# Autodesk Inventor assembly: main climber
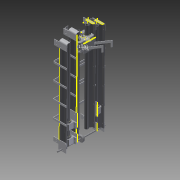
[picture p0: Inventor's stored thumbnail of the model, 180x180]
Saved by Autodesk Inventor 2013 (Build 170138000, 138)
## iProperties
Created: 2013-01-25
Part Number: main climber
Document SubType Name: Assembly
Designer: Arpan
Mass: 3389.77 g
Surface Area: 12723.3 cm^2
Volume: 2953.27 cm^3
Density: 1.1478 g/cm^3
Author: Arpan
## Documents named in this file (18)
- C:\Users\Arpan\Documents\GitHub\frc2013CAD\Cimber actual\main climber.iam
- C:\Users\Arpan\Documents\GitHub\frc2013CAD\Cimber actual\Shaft 26 inch.ipt
- C:\Users\Arpan\Documents\GitHub\frc2013CAD\Cimber actual\Bearing Block long style.iam
- C:\Users\Arpan\Documents\GitHub\frc2013CAD\Cimber actual\hook mount plate.ipt
- C:\Users\Arpan\Documents\GitHub\frc2013CAD\Cimber actual\tie-together tier 1.ipt
- C:\Users\Arpan\Documents\GitHub\frc2013CAD\Cimber actual\endstop.ipt
- C:\Users\Arpan\Documents\GitHub\frc2013CAD\Cimber actual\hook faceplate.ipt
- C:\Users\Arpan\Documents\GitHub\frc2013CAD\Cimber actual\hook.ipt
- C:\Users\Arpan\Documents\GitHub\frc2013CAD\Cimber actual\face mount.ipt
- C:\Users\Arpan\Documents\GitHub\frc2013CAD\Cimber actual\bearing block short style.iam
- C:\Users\Arpan\Documents\GitHub\frc2013CAD\Cimber actual\upper face mount.ipt
- C:\Users\Arpan\Documents\GitHub\frc2013CAD\Cimber actual\tie-together tier 2.ipt
- C:\Users\Arpan\Documents\GitHub\frc2013CAD\Cimber actual\arm mout.ipt
- C:\Users\Arpan\Documents\GitHub\frc2013CAD\Cimber actual\14 inch shaft.ipt
- C:\Users\Arpan\Documents\GitHub\frc2013CAD\Cimber actual\rough pulley.ipt
- C:\Users\Arpan\Documents\GitHub\frc2013CAD\Cimber actual\hook mount plate 2.ipt
- C:\Users\Arpan\Documents\GitHub\frc2013CAD\Cimber actual\endstop 2.ipt
- C:\Users\Arpan\Documents\GitHub\frc2013CAD\Cimber actual\pulley mount.ipt
## Components (36 placed, 17 different names)
1. Shaft 26 inch:1 — Flush:1, Angle:1, Mate:2, Flush:2, Angle:2, Mate:25, Mate:26, Mate:27, Mate:28, Mate:29, Mate:30, Mate:31, Mate:32, Mate:33, Mate:38, Mate:39, Mate:40, Mate:103, Flush:31, Mate:104, Mate:109, Mate:110, Mate:111
2. Shaft 26 inch:2 — Flush:1, Angle:1, Mate:1, Flush:2, Flush:7, Mate:10, Mate:11, Mate:37, Flush:15, Flush:16, Mate:48, Mate:106, Mate:107
3. Bearing Block long style:1 [sub-assembly] — Mate:1, Mate:3, Flush:3
4. Bearing Block long style:2 [sub-assembly] — Mate:2, Mate:3, Angle:2, Flush:3, Mate:98, Flush:25, Flush:26
5. hook mount plate:1 — Mate:98, Mate:99, Flush:25, Flush:26, Flush:27, Mate:100, Flush:28, Mate:101, Flush:29
6. endstop:2 — Flush:7, Mate:10, Mate:11, Mate:116, Flush:35, Flush:36
7. hook faceplate:1 — Mate:20, Mate:21, Mate:22, Flush:13, Flush:14, Mate:23, Mate:99, Mate:101, Flush:29, Mate:102, Flush:30
8. hook:1 — Mate:22, Flush:14, Mate:102
9. hook:2 — Mate:20, Mate:21, Flush:13, Mate:23
10. tie-together tier 1:1 — Mate:25, Mate:26, Mate:27
11. tie-together tier 1:2 — Mate:28, Mate:29, Mate:30
12. tie-together tier 1:3 — Mate:31, Mate:32, Mate:33
13. face mount:1 — Mate:37, Flush:15, Flush:16, Mate:43, Mate:84, Mate:85, Mate:118, Flush:37, Flush:38
14. face mount:2 — Mate:38, Mate:39, Mate:40
15. bearing block short style:2 [sub-assembly] — Mate:43, Flush:19, Mate:84, Mate:85, Flush:23
16. bearing block short style:3 [sub-assembly] — Mate:64, Angle:3, Mate:105
17. bearing block short style:4 [sub-assembly] — Mate:48, Flush:19, Mate:65, Mate:108
18. Shaft 26 inch:3 — Mate:65, Angle:4, Flush:20, Mate:67, Mate:68, Flush:22, Mate:78, Mate:79, Mate:80, Mate:82, Mate:83, Flush:23, Mate:88, Mate:89, Mate:117
19. Shaft 26 inch:4 — Mate:64, Angle:3, Angle:4, Flush:20, Mate:76, Mate:77, Mate:86, Mate:87, Mate:90, Mate:91, Mate:112, Mate:113, Mate:114
20. endstop:3 — Mate:67, Mate:68, Flush:22
21. tie-together tier 2:2 — Mate:76, Mate:77, Mate:78, Mate:117
22. tie-together tier 2:3 — Mate:79, Mate:80
23. tie-together tier 2:4 — Mate:82, Mate:83
24. tie-together tier 2:5 — Mate:86, Mate:87
25. arm mout:1 — Mate:90, Mate:91, Mate:92
26. arm mout:2 — Mate:88, Mate:89, Flush:24, Mate:96
27. 14 inch shaft:1 — Mate:92, Flush:24, Mate:93
28. rough pulley:1 — Mate:93, Mate:96
29. hook mount plate 2:1 — Flush:27, Mate:100, Flush:28, Flush:30
30. upper face mount:1 — Mate:103, Flush:31, Mate:104, Mate:105
31. upper face mount:2 — Mate:106, Mate:107, Mate:108
32. endstop 2:1 — Mate:112, Mate:113, Mate:114, Mate:115, Flush:33, Flush:34
33. endstop 2:2 — Mate:109, Mate:110, Mate:111
34. pulley mount:2 — Mate:115, Flush:33, Flush:34
35. pulley mount:3 — Mate:116, Flush:35, Flush:36
36. pulley mount:4 — Mate:118, Flush:37, Flush:38
## Relationships (97: Mate 67, Flush 26, Angle 4)
- Flush:1: Shaft 26 inch:1 ↔ Shaft 26 inch:2
- Angle:1 (180 deg): Shaft 26 inch:1 ↔ Shaft 26 inch:2
- Mate:1: Shaft 26 inch:2 ↔ Bearing Block long style:1
- Mate:2: Shaft 26 inch:1 ↔ Bearing Block long style:2
- Mate:3 (12.7 mm): Bearing Block long style:1 ↔ Bearing Block long style:2
- Flush:2: Shaft 26 inch:1 ↔ Shaft 26 inch:2
- Angle:2 (0 deg): Shaft 26 inch:1 ↔ Bearing Block long style:2
- Flush:3: Bearing Block long style:1 ↔ Bearing Block long style:2
- Flush:7: Shaft 26 inch:2 ↔ endstop:2
- Mate:10: Shaft 26 inch:2 ↔ endstop:2
- Mate:11: Shaft 26 inch:2 ↔ endstop:2
- Mate:20: hook faceplate:1 ↔ hook:2
- Mate:21 (-26.1747 mm): hook faceplate:1 ↔ hook:2
- Mate:22 (26.1874 mm): hook faceplate:1 ↔ hook:1
- Flush:13 (6.35 mm): hook faceplate:1 ↔ hook:2
- Flush:14 (6.35 mm): hook faceplate:1 ↔ hook:1
- Mate:23 (26.1658 mm): hook faceplate:1 ↔ hook:2
- Mate:25: Shaft 26 inch:1 ↔ tie-together tier 1:1
- Mate:26: Shaft 26 inch:1 ↔ tie-together tier 1:1
- Mate:27: Shaft 26 inch:1 ↔ tie-together tier 1:1
- Mate:28: Shaft 26 inch:1 ↔ tie-together tier 1:2
- Mate:29: Shaft 26 inch:1 ↔ tie-together tier 1:2
- Mate:30: Shaft 26 inch:1 ↔ tie-together tier 1:2
- Mate:31: Shaft 26 inch:1 ↔ tie-together tier 1:3
- Mate:32: Shaft 26 inch:1 ↔ tie-together tier 1:3
- Mate:33: Shaft 26 inch:1 ↔ tie-together tier 1:3
- Mate:37: Shaft 26 inch:2 ↔ face mount:1
- Mate:38: Shaft 26 inch:1 ↔ face mount:2
- Flush:15 (-15.24 mm): Shaft 26 inch:2 ↔ face mount:1
- Flush:16 (-12.688 mm): Shaft 26 inch:2 ↔ face mount:1
- Mate:39: Shaft 26 inch:1 ↔ face mount:2
- Mate:40: Shaft 26 inch:1 ↔ face mount:2
- Mate:43: face mount:1 ↔ bearing block short style:2
- Mate:48 (3.175 mm): Shaft 26 inch:2 ↔ bearing block short style:4
- Flush:19: bearing block short style:2 ↔ bearing block short style:4
- Mate:64: bearing block short style:3 ↔ Shaft 26 inch:4
- Mate:65: bearing block short style:4 ↔ Shaft 26 inch:3
- Angle:3 (180 deg): bearing block short style:3 ↔ Shaft 26 inch:4
- Angle:4 (180 deg): Shaft 26 inch:3 ↔ Shaft 26 inch:4
- Flush:20: Shaft 26 inch:3 ↔ Shaft 26 inch:4
- Mate:67: Shaft 26 inch:3 ↔ endstop:3
- Mate:68: Shaft 26 inch:3 ↔ endstop:3
- Flush:22: Shaft 26 inch:3 ↔ endstop:3
- Mate:76: Shaft 26 inch:4 ↔ tie-together tier 2:2
- Mate:77: Shaft 26 inch:4 ↔ tie-together tier 2:2
- Mate:78: Shaft 26 inch:3 ↔ tie-together tier 2:2
- Mate:79: Shaft 26 inch:3 ↔ tie-together tier 2:3
- Mate:80: Shaft 26 inch:3 ↔ tie-together tier 2:3
- Mate:82: Shaft 26 inch:3 ↔ tie-together tier 2:4
- Mate:83: Shaft 26 inch:3 ↔ tie-together tier 2:4
- Mate:84: face mount:1 ↔ bearing block short style:2
- Mate:85: face mount:1 ↔ bearing block short style:2
- Flush:23: bearing block short style:2 ↔ Shaft 26 inch:3
- Mate:86: Shaft 26 inch:4 ↔ tie-together tier 2:5
- Mate:87: Shaft 26 inch:4 ↔ tie-together tier 2:5
- Mate:88: Shaft 26 inch:3 ↔ arm mout:2
- Mate:89: Shaft 26 inch:3 ↔ arm mout:2
- Mate:90: Shaft 26 inch:4 ↔ arm mout:1
- Mate:91: Shaft 26 inch:4 ↔ arm mout:1
- Mate:92: arm mout:1 ↔ 14 inch shaft:1
- Flush:24 (-33.1 mm): arm mout:2 ↔ 14 inch shaft:1
- Mate:93: 14 inch shaft:1 ↔ rough pulley:1
- Mate:96 (135.1788 mm): arm mout:2 ↔ rough pulley:1
- Mate:98: Bearing Block long style:2 ↔ hook mount plate:1
- Mate:99: hook mount plate:1 ↔ hook faceplate:1
- Flush:25: Bearing Block long style:2 ↔ hook mount plate:1
- Flush:26 (-12.7 mm): Bearing Block long style:2 ↔ hook mount plate:1
- Flush:27: hook mount plate:1 ↔ hook mount plate 2:1
- Mate:100: hook mount plate:1 ↔ hook mount plate 2:1
- Flush:28: hook mount plate:1 ↔ hook mount plate 2:1
- Mate:101: hook mount plate:1 ↔ hook faceplate:1
- Flush:29: hook mount plate:1 ↔ hook faceplate:1
- Mate:102: hook faceplate:1 ↔ hook:1
- Flush:30 (-38.1 mm): hook faceplate:1 ↔ hook mount plate 2:1
- Mate:103: Shaft 26 inch:1 ↔ upper face mount:1
- Flush:31 (-12.7 mm): Shaft 26 inch:1 ↔ upper face mount:1
- Mate:104: Shaft 26 inch:1 ↔ upper face mount:1
- Mate:105: bearing block short style:3 ↔ upper face mount:1
- Mate:106: Shaft 26 inch:2 ↔ upper face mount:2
- Mate:107: Shaft 26 inch:2 ↔ upper face mount:2
- Mate:108: bearing block short style:4 ↔ upper face mount:2
- Mate:109: Shaft 26 inch:1 ↔ endstop 2:2
- Mate:110: Shaft 26 inch:1 ↔ endstop 2:2
- Mate:111: Shaft 26 inch:1 ↔ endstop 2:2
- Mate:112: Shaft 26 inch:4 ↔ endstop 2:1
- Mate:113: Shaft 26 inch:4 ↔ endstop 2:1
- Mate:114: Shaft 26 inch:4 ↔ endstop 2:1
- Mate:115: endstop 2:1 ↔ pulley mount:2
- Flush:33: endstop 2:1 ↔ pulley mount:2
- Flush:34: endstop 2:1 ↔ pulley mount:2
- Mate:116: endstop:2 ↔ pulley mount:3
- Flush:35: endstop:2 ↔ pulley mount:3
- Flush:36: endstop:2 ↔ pulley mount:3
- Mate:117: Shaft 26 inch:3 ↔ tie-together tier 2:2
- Mate:118: face mount:1 ↔ pulley mount:4
- Flush:37: face mount:1 ↔ pulley mount:4
- Flush:38: face mount:1 ↔ pulley mount:4
